# Autodesk Inventor assembly: IR linear array assembly
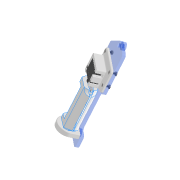
[picture p0: Inventor's stored thumbnail of the model, 180x180]
Saved by Autodesk Inventor 2020 (Build 240168000, 168)
## iProperties
Created: 2020-09-01
Part Number: IR linear array assembly
Document SubType Name: Assembly
Designer: ferrerx
Author: ferrerx
## Documents named in this file (13)
- C:\Users\ferrerx\Desktop\Prieto-Godino Lab\Drosophila Larvae Behavioural Device\Device design V3\Inventor Assembly\IR linear array assembly.iam
- C:\Users\ferrerx\Desktop\Prieto-Godino Lab\Drosophila Larvae Behavioural Device\Device design V3\Inventor Assembly\Acrylic base light source.ipt
- C:\Users\ferrerx\Desktop\Prieto-Godino Lab\Drosophila Larvae Behavioural Device\Device design V3\Inventor Assembly\Micro servo holder.ipt
- C:\Users\ferrerx\Desktop\Prieto-Godino Lab\Drosophila Larvae Behavioural Device\Device design V3\Inventor Assembly\LED linear array holder.ipt
- C:\Users\ferrerx\Desktop\Prieto-Godino Lab\Drosophila Larvae Behavioural Device\Device design V3\Inventor Assembly\MG90s_servo.ipt
- C:\Users\ferrerx\Desktop\Prieto-Godino Lab\Drosophila Larvae Behavioural Device\Device design V3\Inventor Assembly\Shaft atachment.ipt
- C:\Users\ferrerx\Desktop\Prieto-Godino Lab\Drosophila Larvae Behavioural Device\Device design V3\Inventor Assembly\M6 spacer.ipt
- C:\Users\ferrerx\Desktop\Prieto-Godino Lab\Drosophila Larvae Behavioural Device\Device design V3\Inventor Assembly\Servo lever.ipt
- C:\Users\ferrerx\Documents\Inventor\Content Center Files\R2020\en-US\BS 4183(1)\BS 4183 - M3(1).ipt
- C:\Users\ferrerx\Documents\Inventor\Content Center Files\R2020\en-US\AS 1427(03)\AS 1427 - M2 x 16(1).ipt
- C:\Users\ferrerx\Documents\Inventor\Content Center Files\R2020\en-US\AS 1427(04)\AS 1427 - M3 x 12(5) I.ipt
- C:\Users\ferrerx\Desktop\Prieto-Godino Lab\Drosophila Larvae Behavioural Device\Device design V3\Inventor Assembly\Bearing.ipt
- C:\Users\ferrerx\Documents\Inventor\Content Center Files\R2020\en-US\AS 1427(03)\AS 1427 - M2 x 8(1).ipt
## Components (27 placed, 12 different names)
1. Acrylic base light source:1 — Mate:1, Mate:2, Mate:3, Mate:4, Mate:5, Mate:6, Mate:11, Mate:12, Mate:13, Mate:14, Mate:23, Mate:26, Mate:32, Mate:33, Mate:34, Mate:35, Mate:36, Mate:39
2. Micro servo holder:1 — Mate:1, Mate:2, Mate:3, Mate:8, Angle:1, Mate:9, Mate:20, Mate:21, Mate:22, Flush:1, Flush:2, Flush:3, Flush:4, Mate:37, Mate:38
3. LED linear array holder:1 — Mate:7, Mate:10, Mate:16, Angle:2, Mate:43
4. MG90s_servo:1 — Mate:8, Angle:1, Mate:9, Mate:15
5. Shaft atachment:1 — Mate:4, Mate:5, Mate:6, Mate:7, Mate:10, Mate:17, Mate:18, Mate:19, Flush:5, Flush:6, Flush:7, Mate:40, Mate:41
6. M6 spacer:1 — Mate:12, Mate:14
7. M6 spacer:2 — Mate:11, Mate:13
8. Servo lever:1 — Mate:15, Mate:16, Angle:2, Mate:42
9. BS 4183 - Metric M3:1 — Mate:25, Mate:39
10. BS 4183 - Metric M3:2 — Mate:24, Mate:26
11. BS 4183 - Metric M3:3 — Mate:27, Mate:33
12. BS 4183 - Metric M3:4 — Mate:28, Mate:32
13. BS 4183 - Metric M3:5 — Mate:29, Mate:34
14. BS 4183 - Metric M3:6 — Mate:31, Mate:35
15. BS 4183 - Metric M3:7 — Mate:30, Mate:36
16. AS 1427 H - Metric M3 x 12:3 — Mate:17, Flush:6, Mate:29
17. AS 1427 H - Metric M3 x 12:1 — Mate:19, Flush:5, Mate:30
18. AS 1427 H - Metric M3 x 12:2 — Mate:18, Flush:7, Mate:31
19. AS 1427 H - Metric M3 x 12:4 — Mate:20, Mate:25, Flush:2
20. AS 1427 H - Metric M3 x 12:5 — Mate:21, Mate:24, Flush:1
21. AS 1427 H - Metric M3 x 12:6 — Mate:23, Flush:4, Mate:28
22. AS 1427 H - Metric M3 x 12:7 — Mate:22, Flush:3, Mate:27
23. AS 1427 - Metric M2 x 16:1 — Mate:37
24. AS 1427 - Metric M2 x 16:2 — Mate:38
25. Bearing:1 — Mate:40, Mate:41
26. AS 1427 - Metric M2 x 8:1 — Mate:42
27. AS 1427 - Metric M2 x 8:2 — Mate:43
## Relationships (52: Mate 43, Flush 7, Angle 2)
- Mate:1: Acrylic base light source:1 ↔ Micro servo holder:1
- Mate:2: Acrylic base light source:1 ↔ Micro servo holder:1
- Mate:3: Acrylic base light source:1 ↔ Micro servo holder:1
- Mate:4: Acrylic base light source:1 ↔ Shaft atachment:1
- Mate:5: Acrylic base light source:1 ↔ Shaft atachment:1
- Mate:6: Acrylic base light source:1 ↔ Shaft atachment:1
- Mate:7: LED linear array holder:1 ↔ Shaft atachment:1
- Mate:8: Micro servo holder:1 ↔ MG90s_servo:1
- Angle:1 (0 deg): Micro servo holder:1 ↔ MG90s_servo:1
- Mate:9: Micro servo holder:1 ↔ MG90s_servo:1
- Mate:10 (1 mm): LED linear array holder:1 ↔ Shaft atachment:1
- Mate:11: Acrylic base light source:1 ↔ M6 spacer:2
- Mate:12: Acrylic base light source:1 ↔ M6 spacer:1
- Mate:13: Acrylic base light source:1 ↔ M6 spacer:2
- Mate:14: Acrylic base light source:1 ↔ M6 spacer:1
- Mate:15: MG90s_servo:1 ↔ Servo lever:1
- Mate:16: LED linear array holder:1 ↔ Servo lever:1
- Angle:2 (0 deg): LED linear array holder:1 ↔ Servo lever:1
- Mate:17: Shaft atachment:1 ↔ AS 1427 H - Metric M3 x 12:3
- Mate:18: Shaft atachment:1 ↔ AS 1427 H - Metric M3 x 12:2
- Mate:19: Shaft atachment:1 ↔ AS 1427 H - Metric M3 x 12:1
- Mate:20: Micro servo holder:1 ↔ AS 1427 H - Metric M3 x 12:4
- Mate:21: Micro servo holder:1 ↔ AS 1427 H - Metric M3 x 12:5
- Mate:22: Micro servo holder:1 ↔ AS 1427 H - Metric M3 x 12:7
- Mate:23: Acrylic base light source:1 ↔ AS 1427 H - Metric M3 x 12:6
- Mate:24: BS 4183 - Metric M3:2 ↔ AS 1427 H - Metric M3 x 12:5
- Mate:25: BS 4183 - Metric M3:1 ↔ AS 1427 H - Metric M3 x 12:4
- Flush:1: Micro servo holder:1 ↔ AS 1427 H - Metric M3 x 12:5
- Flush:2: Micro servo holder:1 ↔ AS 1427 H - Metric M3 x 12:4
- Flush:3: Micro servo holder:1 ↔ AS 1427 H - Metric M3 x 12:7
- Flush:4: Micro servo holder:1 ↔ AS 1427 H - Metric M3 x 12:6
- Flush:5: Shaft atachment:1 ↔ AS 1427 H - Metric M3 x 12:1
- Flush:6: Shaft atachment:1 ↔ AS 1427 H - Metric M3 x 12:3
- Flush:7: Shaft atachment:1 ↔ AS 1427 H - Metric M3 x 12:2
- Mate:26: Acrylic base light source:1 ↔ BS 4183 - Metric M3:2
- Mate:27: BS 4183 - Metric M3:3 ↔ AS 1427 H - Metric M3 x 12:7
- Mate:28: BS 4183 - Metric M3:4 ↔ AS 1427 H - Metric M3 x 12:6
- Mate:29: BS 4183 - Metric M3:5 ↔ AS 1427 H - Metric M3 x 12:3
- Mate:30: BS 4183 - Metric M3:7 ↔ AS 1427 H - Metric M3 x 12:1
- Mate:31: BS 4183 - Metric M3:6 ↔ AS 1427 H - Metric M3 x 12:2
- Mate:32: Acrylic base light source:1 ↔ BS 4183 - Metric M3:4
- Mate:33: Acrylic base light source:1 ↔ BS 4183 - Metric M3:3
- Mate:34: Acrylic base light source:1 ↔ BS 4183 - Metric M3:5
- Mate:35: Acrylic base light source:1 ↔ BS 4183 - Metric M3:6
- Mate:36: Acrylic base light source:1 ↔ BS 4183 - Metric M3:7
- Mate:37: Micro servo holder:1 ↔ AS 1427 - Metric M2 x 16:1
- Mate:38: Micro servo holder:1 ↔ AS 1427 - Metric M2 x 16:2
- Mate:39: Acrylic base light source:1 ↔ BS 4183 - Metric M3:1
- Mate:40: Shaft atachment:1 ↔ Bearing:1
- Mate:41: Shaft atachment:1 ↔ Bearing:1
- Mate:42: Servo lever:1 ↔ AS 1427 - Metric M2 x 8:1
- Mate:43: LED linear array holder:1 ↔ AS 1427 - Metric M2 x 8:2
